# Autodesk Inventor assembly: Right Hook Whole Assembly
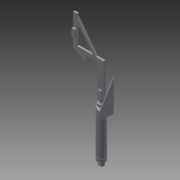
[picture p0: Inventor's stored thumbnail of the model, 180x180]
Saved by Autodesk Inventor 2013 (Build 170138000, 138)
## iProperties
Created: 2013-03-16
Part Number: Right Hook Whole Assembly
Document SubType Name: Assembly
Designer: Arpan
Author: Arpan
## Documents named in this file (4)
- C:\Users\Arpan\Documents\GitHub\frc2013CAD\Right Hook Whole Assembly.iam
- C:\Users\Arpan\Documents\GitHub\frc2013CAD\Midwest Climber\Right Hook Encoder Assembly.iam
- C:\Users\Arpan\Documents\GitHub\frc2013CAD\Midwest Climber\Piston Bracket Assembly.iam
- C:\Users\Arpan\Documents\GitHub\frc2013CAD\Midwest Climber\Ninja cylinder support bracket.ipt
## Components (3 placed, 3 different names)
1. Right Hook Encoder Assembly:1 [sub-assembly] — Angle:1, Angle:2, Mate:1, Mate:2
2. Piston Bracket Assembly:1 [sub-assembly] — Angle:1, Angle:2, Mate:1, Mate:2, Flush:1, Mate:3, Flush:2
3. Ninja cylinder support bracket:1 — Flush:1, Mate:3, Flush:2
## Relationships (7: Mate 3, Angle 2, Flush 2)
- Angle:1 (0 deg): Right Hook Encoder Assembly:1 ↔ Piston Bracket Assembly:1
- Angle:2 (0 deg): Right Hook Encoder Assembly:1 ↔ Piston Bracket Assembly:1
- Mate:1: Right Hook Encoder Assembly:1 ↔ Piston Bracket Assembly:1
- Mate:2: Right Hook Encoder Assembly:1 ↔ Piston Bracket Assembly:1
- Flush:1: Piston Bracket Assembly:1 ↔ Ninja cylinder support bracket:1
- Mate:3: Piston Bracket Assembly:1 ↔ Ninja cylinder support bracket:1
- Flush:2: Piston Bracket Assembly:1 ↔ Ninja cylinder support bracket:1
